# Autodesk Inventor assembly: x2010-8-FIRSTwheel
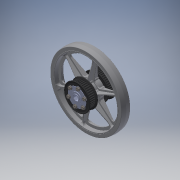
[picture p0: Inventor's stored thumbnail of the model, 180x180]
Saved by Autodesk Inventor 2016 (Build 200138000, 138)
## iProperties
Company: Unknown
Created: 2016-01-13
Part Number: x2010-8-FIRSTwheel
Description: Unknown
Document SubType Name: Assembly
Designer: Douglas
Sending System: Unknown
Preprocessor: XStep 1.0
Title: //Amserv/amserver/AndyMark/Products/Wheels Solid/FIRST Wheel 2010 8 inch/2010 8 wheel.stp
Author: Unknown
Revision Number: NONE
## Documents named in this file (7)
- D:\Douglas\Documents\Git\2016-Robot-CAD\Inventor\PARTS\x2010-8-FIRSTwheel.iam
- D:\Douglas\Documents\Git\2016-Robot-CAD\Inventor\PARTS\2010 8 tread.ipt
- D:\Douglas\Documents\Git\2016-Robot-CAD\Inventor\PARTS\2010 8 hub.ipt
- D:\Douglas\Documents\Git\2016-Robot-CAD\Inventor\Chassis\42 tooth HTD Pulley half 2014.ipt
- D:\Douglas\Documents\Git\2016-Robot-CAD\Inventor\Chassis\500EX Hex Hub.ipt
- D:\Douglas\Documents\Git\2016-Robot-CAD\Inventor\Chassis\am-1305 500 Hex Spacer.ipt
- D:\Douglas\Documents\Git\2016-Robot-CAD\Inventor\Chassis\10-24 Hex Washer Rolling x 1.25_93882A213.ipt
## Components (20 placed, 6 different names)
1. 2010 8 tread — Mate:4, Flush:1
2. 2010 8 hub — Mate:4, Flush:1, Mate:5, Mate:6, Mate:7, Mate:11, Mate:12, Mate:13
3. 42 tooth HTD Pulley half 2014:1 — Mate:1, Mate:2, Mate:3, Mate:5, Mate:6, Mate:7
4. 42 tooth HTD Pulley half 2014:2 — Mate:1, Mate:2, Mate:3, Mate:14, Mate:15, Mate:16
5. 42 tooth HTD Pulley half 2014:3 — Mate:19, Mate:20, Mate:21, Mate:22, Mate:23, Mate:24, Mate:25, Mate:26, Mate:27, Mate:28, Mate:29, Mate:30, Mate:43
6. 42 tooth HTD Pulley half 2014:4 — Mate:11, Mate:12, Mate:13
7. 500EX Hex Hub:1 — Mate:14, Mate:15, Mate:16, Mate:31, Mate:32, Mate:33, Mate:34, Mate:35, Mate:36, Mate:37, Mate:38, Mate:39, Mate:40, Mate:41, Mate:42
8. am-1305 500 Hex Spacer:1 — Mate:43
9. 10-24 Hex Washer Rolling x 1.25_93882A213:1 — Mate:19, Mate:20
10. 10-24 Hex Washer Rolling x 1.25_93882A213:2 — Mate:21, Mate:22
11. 10-24 Hex Washer Rolling x 1.25_93882A213:3 — Mate:23, Mate:24
12. 10-24 Hex Washer Rolling x 1.25_93882A213:4 — Mate:29, Mate:30
13. 10-24 Hex Washer Rolling x 1.25_93882A213:5 — Mate:41, Mate:42
14. 10-24 Hex Washer Rolling x 1.25_93882A213:6 — Mate:39, Mate:40
15. 10-24 Hex Washer Rolling x 1.25_93882A213:7 — Mate:37, Mate:38
16. 10-24 Hex Washer Rolling x 1.25_93882A213:8 — Mate:25, Mate:26
17. 10-24 Hex Washer Rolling x 1.25_93882A213:9 — Mate:35, Mate:36
18. 10-24 Hex Washer Rolling x 1.25_93882A213:10 — Mate:33, Mate:34
19. 10-24 Hex Washer Rolling x 1.25_93882A213:11 — Mate:31, Mate:32
20. 10-24 Hex Washer Rolling x 1.25_93882A213:12 — Mate:27, Mate:28
## Relationships (42: Mate 41, Flush 1)
- Mate:1: 42 tooth HTD Pulley half 2014:1 ↔ 42 tooth HTD Pulley half 2014:2
- Mate:2: 42 tooth HTD Pulley half 2014:1 ↔ 42 tooth HTD Pulley half 2014:2
- Mate:3: 42 tooth HTD Pulley half 2014:1 ↔ 42 tooth HTD Pulley half 2014:2
- Mate:4: 2010 8 tread ↔ 2010 8 hub
- Flush:1: 2010 8 tread ↔ 2010 8 hub
- Mate:5: 2010 8 hub ↔ 42 tooth HTD Pulley half 2014:1
- Mate:6: 2010 8 hub ↔ 42 tooth HTD Pulley half 2014:1
- Mate:7: 2010 8 hub ↔ 42 tooth HTD Pulley half 2014:1
- [Mate]: 42 tooth HTD Pulley half 2014:3 ↔ 42 tooth HTD Pulley half 2014:4
- [Mate]: 42 tooth HTD Pulley half 2014:3 ↔ 42 tooth HTD Pulley half 2014:4
- [Mate]: 42 tooth HTD Pulley half 2014:3 ↔ 42 tooth HTD Pulley half 2014:4
- Mate:11: 2010 8 hub ↔ 42 tooth HTD Pulley half 2014:4
- Mate:12: 2010 8 hub ↔ 42 tooth HTD Pulley half 2014:4
- Mate:13: 2010 8 hub ↔ 42 tooth HTD Pulley half 2014:4
- Mate:14: 42 tooth HTD Pulley half 2014:2 ↔ 500EX Hex Hub:1
- Mate:15: 42 tooth HTD Pulley half 2014:2 ↔ 500EX Hex Hub:1
- Mate:16: 42 tooth HTD Pulley half 2014:2 ↔ 500EX Hex Hub:1
- Mate:19: 42 tooth HTD Pulley half 2014:3 ↔ 10-24 Hex Washer Rolling x 1.25_93882A213:1
- Mate:20: 42 tooth HTD Pulley half 2014:3 ↔ 10-24 Hex Washer Rolling x 1.25_93882A213:1
- Mate:21: 42 tooth HTD Pulley half 2014:3 ↔ 10-24 Hex Washer Rolling x 1.25_93882A213:2
- Mate:22: 42 tooth HTD Pulley half 2014:3 ↔ 10-24 Hex Washer Rolling x 1.25_93882A213:2
- Mate:23: 42 tooth HTD Pulley half 2014:3 ↔ 10-24 Hex Washer Rolling x 1.25_93882A213:3
- Mate:24: 42 tooth HTD Pulley half 2014:3 ↔ 10-24 Hex Washer Rolling x 1.25_93882A213:3
- Mate:25: 42 tooth HTD Pulley half 2014:3 ↔ 10-24 Hex Washer Rolling x 1.25_93882A213:8
- Mate:26: 42 tooth HTD Pulley half 2014:3 ↔ 10-24 Hex Washer Rolling x 1.25_93882A213:8
- Mate:27: 42 tooth HTD Pulley half 2014:3 ↔ 10-24 Hex Washer Rolling x 1.25_93882A213:12
- Mate:28: 42 tooth HTD Pulley half 2014:3 ↔ 10-24 Hex Washer Rolling x 1.25_93882A213:12
- Mate:29: 42 tooth HTD Pulley half 2014:3 ↔ 10-24 Hex Washer Rolling x 1.25_93882A213:4
- Mate:30: 42 tooth HTD Pulley half 2014:3 ↔ 10-24 Hex Washer Rolling x 1.25_93882A213:4
- Mate:31: 500EX Hex Hub:1 ↔ 10-24 Hex Washer Rolling x 1.25_93882A213:11
- Mate:32: 500EX Hex Hub:1 ↔ 10-24 Hex Washer Rolling x 1.25_93882A213:11
- Mate:33: 500EX Hex Hub:1 ↔ 10-24 Hex Washer Rolling x 1.25_93882A213:10
- Mate:34: 500EX Hex Hub:1 ↔ 10-24 Hex Washer Rolling x 1.25_93882A213:10
- Mate:35: 500EX Hex Hub:1 ↔ 10-24 Hex Washer Rolling x 1.25_93882A213:9
- Mate:36: 500EX Hex Hub:1 ↔ 10-24 Hex Washer Rolling x 1.25_93882A213:9
- Mate:37: 500EX Hex Hub:1 ↔ 10-24 Hex Washer Rolling x 1.25_93882A213:7
- Mate:38: 500EX Hex Hub:1 ↔ 10-24 Hex Washer Rolling x 1.25_93882A213:7
- Mate:39: 500EX Hex Hub:1 ↔ 10-24 Hex Washer Rolling x 1.25_93882A213:6
- Mate:40: 500EX Hex Hub:1 ↔ 10-24 Hex Washer Rolling x 1.25_93882A213:6
- Mate:41: 500EX Hex Hub:1 ↔ 10-24 Hex Washer Rolling x 1.25_93882A213:5
- Mate:42: 500EX Hex Hub:1 ↔ 10-24 Hex Washer Rolling x 1.25_93882A213:5
- Mate:43: 42 tooth HTD Pulley half 2014:3 ↔ am-1305 500 Hex Spacer:1
## Named parameters: d8_d0 = 0 mm, d9_d1 = 0 mm, d10_d2 = 0 mm
